# Autodesk Inventor assembly: Walls + Top Lid
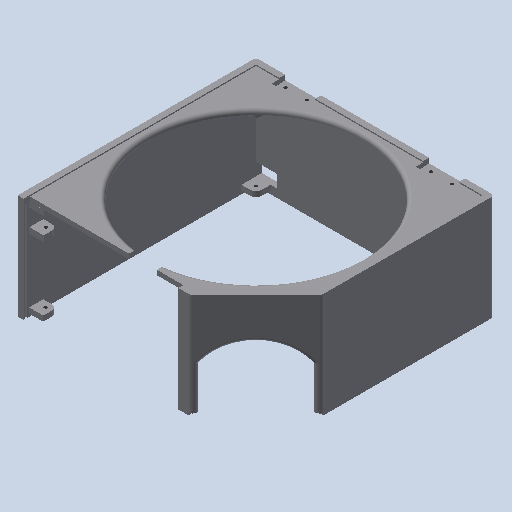
[picture p0: Inventor's stored thumbnail of the model, 512x512]
Saved by Autodesk Inventor 2022 (Build 260153000, 153)
## iProperties
Created: 2023-03-11
Part Number: Walls + Top Lid
Document SubType Name: Assembly
Designer: zarek
Author: zarek
## Documents named in this file (3)
- C:\Users\zarek\OneDrive\Desktop\Random New Stuff\SPB\Box Walls + Top Lid.iam
- C:\Users\zarek\OneDrive\Desktop\Random New Stuff\SPB\Box_Walls_2 - Copy.ipt
- C:\Users\zarek\OneDrive\Desktop\Random New Stuff\SPB\Lid_Inside_Base.ipt
## Components (2 placed, 2 different names)
1. Box_Walls_2 - Copy:1 — Mate:1, Mate:2
2. Lid_Inside_Base:2 — Mate:1, Mate:2
## Relationships (2: Mate 2)
- Mate:1: Box_Walls_2 - Copy:1 ↔ Lid_Inside_Base:2
- Mate:2: Box_Walls_2 - Copy:1 ↔ Lid_Inside_Base:2
